# Autodesk Inventor assembly: VerticalAssembly
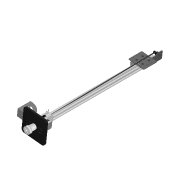
[picture p0: Inventor's stored thumbnail of the model, 180x180]
Saved by Autodesk Inventor 2020.3 (Build 243373000, 373)
## iProperties
Created: 2021-08-03
Part Number: VerticalAssembly
Document SubType Name: Assembly
Designer: justi
Mass: 692.174 g
Surface Area: 2682.96 cm^2
Volume: 292.624 cm^3
Density: 2.3654 g/cm^3
Author: justi
## Documents named in this file (23)
- F:\UQ Engineering\2021 ~ 5th Year\Semester 2\METR4911-THESIS\FarmBot CAD\FarmBotV1\VerticalAssembly.iam
- F:\UQ Engineering\2021 ~ 5th Year\Semester 2\METR4911-THESIS\FarmBot CAD\FarmBotV1\LinearRail\20x40x597mm.ipt
- F:\UQ Engineering\2021 ~ 5th Year\Semester 2\METR4911-THESIS\FarmBot CAD\FarmBotV1\VerticalSlidingCart.iam
- F:\UQ Engineering\2021 ~ 5th Year\Semester 2\METR4911-THESIS\FarmBot CAD\FarmBotV1\ActuatorPulleyPlate.ipt
- F:\UQ Engineering\2021 ~ 5th Year\Semester 2\METR4911-THESIS\FarmBot CAD\FarmBotV1\VSlotHardware\Idler pulley kit.iam
- F:\UQ Engineering\2021 ~ 5th Year\Semester 2\METR4911-THESIS\FarmBot CAD\FarmBotV1\Rework+Simple+25_1+Cycloidal+Actuator\files\sim_nema_17\Workspaces\Workspace\robot arm\Motor_paso.ipt
- F:\UQ Engineering\2021 ~ 5th Year\Semester 2\METR4911-THESIS\FarmBot CAD\FarmBotV1\GT2 Timing Pulley, Configurable, 20T W6 B5.iam
- F:\UQ Engineering\2021 ~ 5th Year\Semester 2\METR4911-THESIS\FarmBot CAD\FarmBotV1\VerticalActuationPlate_V2.ipt
- F:\UQ Engineering\2021 ~ 5th Year\Semester 2\METR4911-THESIS\FarmBot CAD\FarmBotV1\VerticalActuationPlate_V2_MIR1.ipt
- F:\UQ Engineering\2021 ~ 5th Year\Semester 2\METR4911-THESIS\FarmBot CAD\FarmBotV1\VerticalActuationMount.ipt
- F:\UQ Engineering\2021 ~ 5th Year\Semester 2\METR4911-THESIS\FarmBot CAD\FarmBotV1\GT2 pulley 60 teeth width 11mm 8mm bore.ipt
- F:\UQ Engineering\2021 ~ 5th Year\Semester 2\METR4911-THESIS\FarmBot CAD\FarmBotV1\CableChainVerticalAxisMount.ipt
- F:\UQ Engineering\2021 ~ 5th Year\Semester 2\METR4911-THESIS\FarmBot CAD\FarmBotV1\CableChainVerticlAxisMount2.ipt
- F:\UQ Engineering\2021 ~ 5th Year\Semester 2\METR4911-THESIS\FarmBot CAD\FarmBotV1\VSlotHardware\V-Wheel Kit.iam
- F:\UQ Engineering\2021 ~ 5th Year\Semester 2\METR4911-THESIS\FarmBot CAD\FarmBotV1\LimitSwitchAssembly.iam
- F:\UQ Engineering\2021 ~ 5th Year\Semester 2\METR4911-THESIS\FarmBot CAD\FarmBotV1\PuleyIdlerHolder.ipt
- F:\UQ Engineering\2021 ~ 5th Year\Semester 2\METR4911-THESIS\FarmBot CAD\FarmBotV1\GT2_TimingBelt Vert.ipt
- F:\UQ Engineering\2021 ~ 5th Year\Semester 2\METR4911-THESIS\FarmBot CAD\FarmBotV1\VerticalAssembly\AIP\FEA\drv0tcd0g.fins
- F:\UQ Engineering\2021 ~ 5th Year\Semester 2\METR4911-THESIS\FarmBot CAD\FarmBotV1\VerticalAssembly\AIP\FEA\drv0tcd0g.fsat
- F:\UQ Engineering\2021 ~ 5th Year\Semester 2\METR4911-THESIS\FarmBot CAD\FarmBotV1\VerticalAssembly\AIP\FEA\drv0tcd1c.ftes
- F:\UQ Engineering\2021 ~ 5th Year\Semester 2\METR4911-THESIS\FarmBot CAD\FarmBotV1\VerticalAssembly\AIP\FEA\drv0tcd1c.fwiz
- F:\UQ Engineering\2021 ~ 5th Year\Semester 2\METR4911-THESIS\FarmBot CAD\FarmBotV1\VerticalAssembly\AIP\FEA\drv0tcd8g.fmsh
- F:\UQ Engineering\2021 ~ 5th Year\Semester 2\METR4911-THESIS\FarmBot CAD\FarmBotV1\VerticalAssembly\AIP\FEA\drv0tcd9c.fres
## Components (18 placed, 16 different names)
1. 20x40x597mm:1 — Mate:8, Mate:9, Mate:41, Mate:42, Mate:43, Mate:50, Mate:55, Mate:82, Mate:83, Mate:84, Flush:1, Mate:86, Flush:88, Mate:88
2. VerticalSlidingCart:1 [sub-assembly] — Mate:8, Mate:9, Mate:67, Mate:68, Mate:69
3. ActuatorPulleyPlate:1 — Mate:82, Mate:83, Mate:84, Flush:1, Mate:85, Flush:89, Mate:90
4. Idler pulley kit:1 [sub-assembly] — Mate:85, Flush:2, Mate:92
5. Motor_paso:1 — Mate:25, Mate:45, Mate:46, Mate:47
6. GT2 Timing Pulley, Configurable, 20T W6 B5:1 [sub-assembly] — Mate:25, Mate:51, Mate:80, Mate:81, Flush:2, Mate:91, Mate:94
7. VerticalActuationPlate_V2:1 — Mate:41, Mate:42, Mate:43, Mate:45, Mate:46, Mate:47, Mate:48, Mate:49, Mate:78
8. VerticalActuationPlate_V2_MIR1:1 — Mate:48, Mate:49, Mate:50, Mate:51, Mate:54, Mate:64, Mate:66, Mate:70, Mate:71, Mate:72, Mate:79, Mate:89, Flush:90
9. VerticalActuationMount:1 — Mate:54, Mate:55, Mate:59, Mate:60, Mate:61, Mate:64, Mate:66
10. GT2 pulley 60 teeth width 11mm 8mm bore:1 — Mate:59, Mate:60, Mate:61
11. CableChainVerticalAxisMount:1 — Mate:67, Mate:68, Mate:69
12. CableChainVerticlAxisMount2:1 — Mate:70, Mate:71, Mate:72
13. V-Wheel Kit:1 [sub-assembly] — Mate:78, Mate:80
14. V-Wheel Kit:2 [sub-assembly] — Mate:79, Mate:81
15. LimitSwitchAssembly:1 [sub-assembly] — Mate:86, Flush:88, Flush:89
16. LimitSwitchAssembly:2 [sub-assembly] — Mate:88, Mate:89, Flush:90
17. PuleyIdlerHolder:1 — Mate:90, Mate:91, Mate:93
18. GT2_TimingBelt Vert:1 — Mate:92, Mate:93, Mate:94
## Relationships (47: Mate 42, Flush 5)
- Mate:8 (1 mm): 20x40x597mm:1 ↔ VerticalSlidingCart:1
- Mate:9: 20x40x597mm:1 ↔ VerticalSlidingCart:1
- Mate:25: Motor_paso:1 ↔ GT2 Timing Pulley, Configurable, 20T W6 B5:1
- Mate:41: 20x40x597mm:1 ↔ VerticalActuationPlate_V2:1
- Mate:42: 20x40x597mm:1 ↔ VerticalActuationPlate_V2:1
- Mate:43: 20x40x597mm:1 ↔ VerticalActuationPlate_V2:1
- Mate:45: Motor_paso:1 ↔ VerticalActuationPlate_V2:1
- Mate:46: Motor_paso:1 ↔ VerticalActuationPlate_V2:1
- Mate:47: Motor_paso:1 ↔ VerticalActuationPlate_V2:1
- Mate:48: VerticalActuationPlate_V2:1 ↔ VerticalActuationPlate_V2_MIR1:1
- Mate:49: VerticalActuationPlate_V2:1 ↔ VerticalActuationPlate_V2_MIR1:1
- Mate:50: 20x40x597mm:1 ↔ VerticalActuationPlate_V2_MIR1:1
- Mate:51: GT2 Timing Pulley, Configurable, 20T W6 B5:1 ↔ VerticalActuationPlate_V2_MIR1:1
- Mate:54: VerticalActuationPlate_V2_MIR1:1 ↔ VerticalActuationMount:1
- Mate:55 (65 mm): 20x40x597mm:1 ↔ VerticalActuationMount:1
- Mate:59: VerticalActuationMount:1 ↔ GT2 pulley 60 teeth width 11mm 8mm bore:1
- Mate:60: VerticalActuationMount:1 ↔ GT2 pulley 60 teeth width 11mm 8mm bore:1
- Mate:61: VerticalActuationMount:1 ↔ GT2 pulley 60 teeth width 11mm 8mm bore:1
- Mate:64: VerticalActuationPlate_V2_MIR1:1 ↔ VerticalActuationMount:1
- Mate:66: VerticalActuationPlate_V2_MIR1:1 ↔ VerticalActuationMount:1
- Mate:67: VerticalSlidingCart:1 ↔ CableChainVerticalAxisMount:1
- Mate:68: VerticalSlidingCart:1 ↔ CableChainVerticalAxisMount:1
- Mate:69: VerticalSlidingCart:1 ↔ CableChainVerticalAxisMount:1
- Mate:70: VerticalActuationPlate_V2_MIR1:1 ↔ CableChainVerticlAxisMount2:1
- Mate:71: VerticalActuationPlate_V2_MIR1:1 ↔ CableChainVerticlAxisMount2:1
- Mate:72: VerticalActuationPlate_V2_MIR1:1 ↔ CableChainVerticlAxisMount2:1
- Mate:78: VerticalActuationPlate_V2:1 ↔ V-Wheel Kit:1
- Mate:79: VerticalActuationPlate_V2_MIR1:1 ↔ V-Wheel Kit:2
- Mate:80: GT2 Timing Pulley, Configurable, 20T W6 B5:1 ↔ V-Wheel Kit:1
- Mate:81: GT2 Timing Pulley, Configurable, 20T W6 B5:1 ↔ V-Wheel Kit:2
- Mate:82: 20x40x597mm:1 ↔ ActuatorPulleyPlate:1
- Mate:83: 20x40x597mm:1 ↔ ActuatorPulleyPlate:1
- Mate:84: 20x40x597mm:1 ↔ ActuatorPulleyPlate:1
- Flush:1 (-45 mm): 20x40x597mm:1 ↔ ActuatorPulleyPlate:1
- Mate:85: ActuatorPulleyPlate:1 ↔ Idler pulley kit:1
- Flush:2: Idler pulley kit:1 ↔ GT2 Timing Pulley, Configurable, 20T W6 B5:1
- Mate:86: 20x40x597mm:1 ↔ LimitSwitchAssembly:1
- Flush:88: 20x40x597mm:1 ↔ LimitSwitchAssembly:1
- Flush:89: ActuatorPulleyPlate:1 ↔ LimitSwitchAssembly:1
- Mate:88: 20x40x597mm:1 ↔ LimitSwitchAssembly:2
- Mate:89: VerticalActuationPlate_V2_MIR1:1 ↔ LimitSwitchAssembly:2
- Flush:90: VerticalActuationPlate_V2_MIR1:1 ↔ LimitSwitchAssembly:2
- Mate:90: ActuatorPulleyPlate:1 ↔ PuleyIdlerHolder:1
- Mate:91: GT2 Timing Pulley, Configurable, 20T W6 B5:1 ↔ PuleyIdlerHolder:1
- Mate:92: Idler pulley kit:1 ↔ GT2_TimingBelt Vert:1
- Mate:93: PuleyIdlerHolder:1 ↔ GT2_TimingBelt Vert:1
- Mate:94: GT2 Timing Pulley, Configurable, 20T W6 B5:1 ↔ GT2_TimingBelt Vert:1
